# Autodesk Inventor assembly: lifterB
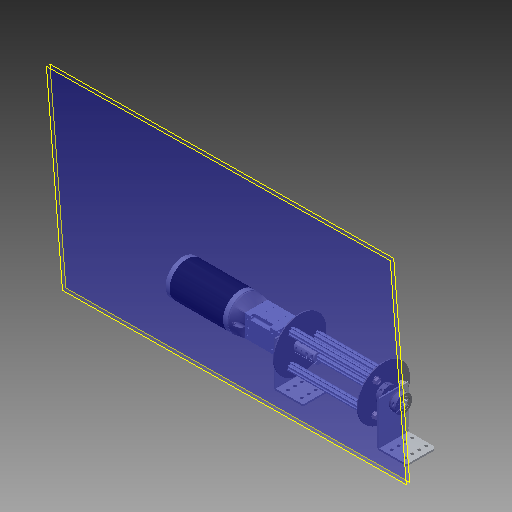
[picture p0: Inventor's stored thumbnail of the model, 512x512]
Saved by Autodesk Inventor 2017 (Build 210142000, 142)
## iProperties
Created: 2017-03-08
Part Number: lifterB
Document SubType Name: Assembly
Designer: kingb
Author: kingb
## Documents named in this file (10)
- C:\Users\admin\Desktop\CAD\lifterB.iam
- C:\Users\admin\Desktop\CAD\spoolEnd.ipt
- C:\Users\admin\Desktop\CAD\spoolChurro.ipt
- C:\Users\admin\Desktop\CAD\FHTS 0.25-20-0.75_FHTS 0.25-20-G-0.75-C.ipt
- C:\Users\admin\Desktop\CAD\Churro 20250.ipt
- C:\Users\admin\Desktop\CAD\FR8ZZ Hex Bearing.ipt
- C:\Users\admin\Desktop\CAD\7552K500_HEXAGONAL-BORE CLAMP-ON SHAFT COLLAR.ipt
- C:\Users\admin\Desktop\CAD\mountedLifterMotor.iam
- C:\Users\admin\Desktop\CAD\217-4008-001 Rev1.ipt
- C:\Users\admin\Desktop\CAD\motorMount.ipt
## Components (22 placed, 9 different names)
1. spoolChurro:1 — Insert:1, Insert:4, Angle:2, Angle:6, Angle:9
2. spoolEnd:1 — Insert:1, Insert:2, Insert:3, Insert:7, Insert:8, Insert:9, Mate:1, Mate:2, Mate:18, Mate:28
3. spoolChurro:2 — Insert:3, Insert:6, Angle:3, Angle:5, Angle:7
4. spoolChurro:3 — Insert:2, Insert:5, Angle:1, Angle:4, Angle:8
5. spoolEnd:2 — Insert:4, Insert:5, Insert:6, Angle:1, Angle:2, Angle:3, Insert:10, Insert:11, Insert:12, Tangent:1, Mate:39
6. FHTS 0.25-20-0.75_FHTS 0.25-20-G-0.75-C:1 — Insert:12, Angle:4
7. FHTS 0.25-20-0.75_FHTS 0.25-20-G-0.75-C:2 — Insert:10, Angle:6
8. FHTS 0.25-20-0.75_FHTS 0.25-20-G-0.75-C:3 — Insert:11, Angle:5
9. FHTS 0.25-20-0.75_FHTS 0.25-20-G-0.75-C:4 — Insert:7, Angle:9
10. FHTS 0.25-20-0.75_FHTS 0.25-20-G-0.75-C:5 — Insert:9, Angle:8
11. FHTS 0.25-20-0.75_FHTS 0.25-20-G-0.75-C:6 — Insert:8, Angle:7
12. Churro 20250:1 — Mate:1, Mate:2, Mate:3, Mate:4, Mate:5, Mate:6, Mate:13, Mate:14, Mate:15, Mate:16, Flush:2, Mate:23, Mate:24, Mate:30, Mate:31, Mate:32, Insert:13
13. FR8ZZ Hex Bearing:1 — Mate:3, Mate:4, Mate:36, Mate:40
14. FR8ZZ Hex Bearing:2 — Mate:5, Mate:6, Mate:34, Mate:37, Mate:38
15. 7552K500_HEXAGONAL-BORE CLAMP-ON SHAFT COLLAR:1 — Mate:13, Mate:14, Mate:40
16. 7552K500_HEXAGONAL-BORE CLAMP-ON SHAFT COLLAR:2 — Mate:15, Mate:16, Mate:18, Mate:37
17. mountedLifterMotor:1 [sub-assembly] — Flush:2, Mate:22, Mate:25, Tangent:2, Insert:13, Mate:38, Angle:11
18. 217-4008-001 Rev1:1 — Mate:24, Mate:25, Flush:4
19. 217-4008-001 Rev1:2 — Mate:22, Mate:23, Flush:4, Mate:28
20. 7552K500_HEXAGONAL-BORE CLAMP-ON SHAFT COLLAR:3 — Mate:30, Mate:31, Mate:39
21. motorMount:1 — Tangent:2, Flush:5, Flush:7, Mate:32, Mate:35, Mate:36
22. motorMount:2 — Flush:5, Flush:7, Mate:34, Mate:35, Angle:11
## Relationships (57: Mate 26, Insert 13, Angle 11, Flush 5, Tangent 2)
- Insert:1: spoolChurro:1 ↔ spoolEnd:1
- Insert:2: spoolEnd:1 ↔ spoolChurro:3
- Insert:3: spoolEnd:1 ↔ spoolChurro:2
- Insert:4: spoolChurro:1 ↔ spoolEnd:2
- Insert:5: spoolChurro:3 ↔ spoolEnd:2
- Insert:6: spoolChurro:2 ↔ spoolEnd:2
- Angle:1 (0 deg): spoolChurro:3 ↔ spoolEnd:2
- Angle:2 (0 deg): spoolChurro:1 ↔ spoolEnd:2
- Angle:3 (0 deg): spoolChurro:2 ↔ spoolEnd:2
- Insert:7: spoolEnd:1 ↔ FHTS 0.25-20-0.75_FHTS 0.25-20-G-0.75-C:4
- Insert:8: spoolEnd:1 ↔ FHTS 0.25-20-0.75_FHTS 0.25-20-G-0.75-C:6
- Insert:9: spoolEnd:1 ↔ FHTS 0.25-20-0.75_FHTS 0.25-20-G-0.75-C:5
- Insert:10: spoolEnd:2 ↔ FHTS 0.25-20-0.75_FHTS 0.25-20-G-0.75-C:2
- Insert:11: spoolEnd:2 ↔ FHTS 0.25-20-0.75_FHTS 0.25-20-G-0.75-C:3
- Insert:12: spoolEnd:2 ↔ FHTS 0.25-20-0.75_FHTS 0.25-20-G-0.75-C:1
- Angle:4 (0 deg): spoolChurro:3 ↔ FHTS 0.25-20-0.75_FHTS 0.25-20-G-0.75-C:1
- Angle:5 (0 deg): spoolChurro:2 ↔ FHTS 0.25-20-0.75_FHTS 0.25-20-G-0.75-C:3
- Angle:6 (0 deg): spoolChurro:1 ↔ FHTS 0.25-20-0.75_FHTS 0.25-20-G-0.75-C:2
- Angle:7 (0 deg): spoolChurro:2 ↔ FHTS 0.25-20-0.75_FHTS 0.25-20-G-0.75-C:6
- Angle:8 (0 deg): spoolChurro:3 ↔ FHTS 0.25-20-0.75_FHTS 0.25-20-G-0.75-C:5
- Angle:9 (0 deg): spoolChurro:1 ↔ FHTS 0.25-20-0.75_FHTS 0.25-20-G-0.75-C:4
- Mate:1: spoolEnd:1 ↔ Churro 20250:1
- Mate:2: spoolEnd:1 ↔ Churro 20250:1
- Angle:10 (0 deg)
- Tangent:1: spoolEnd:2
- Flush:1 (-6.35 mm)
- Mate:3: Churro 20250:1 ↔ FR8ZZ Hex Bearing:1
- Mate:4: Churro 20250:1 ↔ FR8ZZ Hex Bearing:1
- Mate:5: Churro 20250:1 ↔ FR8ZZ Hex Bearing:2
- Mate:6: Churro 20250:1 ↔ FR8ZZ Hex Bearing:2
- Mate:13: Churro 20250:1 ↔ 7552K500_HEXAGONAL-BORE CLAMP-ON SHAFT COLLAR:1
- Mate:14: Churro 20250:1 ↔ 7552K500_HEXAGONAL-BORE CLAMP-ON SHAFT COLLAR:1
- Mate:15: Churro 20250:1 ↔ 7552K500_HEXAGONAL-BORE CLAMP-ON SHAFT COLLAR:2
- Mate:16: Churro 20250:1 ↔ 7552K500_HEXAGONAL-BORE CLAMP-ON SHAFT COLLAR:2
- Mate:18: spoolEnd:1 ↔ 7552K500_HEXAGONAL-BORE CLAMP-ON SHAFT COLLAR:2
- Flush:2: Churro 20250:1 ↔ mountedLifterMotor:1
- Mate:22: mountedLifterMotor:1 ↔ 217-4008-001 Rev1:2
- Mate:23: Churro 20250:1 ↔ 217-4008-001 Rev1:2
- Mate:24: Churro 20250:1 ↔ 217-4008-001 Rev1:1
- Mate:25: mountedLifterMotor:1 ↔ 217-4008-001 Rev1:1
- Flush:4: 217-4008-001 Rev1:1 ↔ 217-4008-001 Rev1:2
- Mate:28: spoolEnd:1 ↔ 217-4008-001 Rev1:2
- Mate:30: Churro 20250:1 ↔ 7552K500_HEXAGONAL-BORE CLAMP-ON SHAFT COLLAR:3
- Mate:31: Churro 20250:1 ↔ 7552K500_HEXAGONAL-BORE CLAMP-ON SHAFT COLLAR:3
- Tangent:2 (31.75 mm): mountedLifterMotor:1 ↔ motorMount:1
- Flush:5: motorMount:1 ↔ motorMount:2
- Flush:7: motorMount:1 ↔ motorMount:2
- Mate:32 (-21.4312 mm): Churro 20250:1 ↔ motorMount:1
- Mate:34: FR8ZZ Hex Bearing:2 ↔ motorMount:2
- Mate:35 (190.5 mm): motorMount:1 ↔ motorMount:2
- Insert:13: Churro 20250:1 ↔ mountedLifterMotor:1
- Mate:36: FR8ZZ Hex Bearing:1 ↔ motorMount:1
- Mate:37: FR8ZZ Hex Bearing:2 ↔ 7552K500_HEXAGONAL-BORE CLAMP-ON SHAFT COLLAR:2
- Mate:38: FR8ZZ Hex Bearing:2 ↔ mountedLifterMotor:1
- Mate:39: spoolEnd:2 ↔ 7552K500_HEXAGONAL-BORE CLAMP-ON SHAFT COLLAR:3
- Mate:40: FR8ZZ Hex Bearing:1 ↔ 7552K500_HEXAGONAL-BORE CLAMP-ON SHAFT COLLAR:1
- Angle:11 (90 deg): mountedLifterMotor:1 ↔ motorMount:2
